# Autodesk Inventor assembly: 1071_assembly
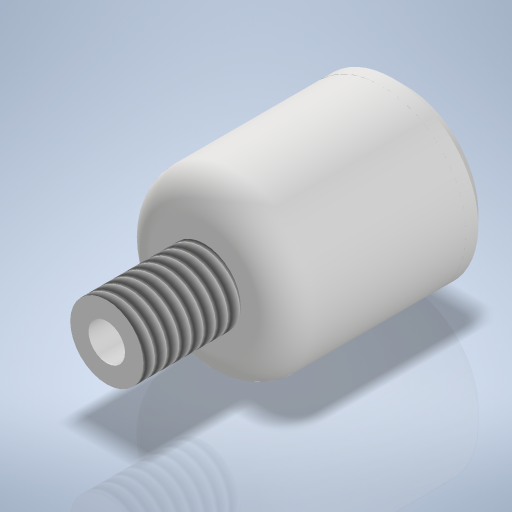
[picture p0: Inventor's stored thumbnail of the model, 512x512]
Saved by Autodesk Inventor 2024 (Build 280153000, 153)
## iProperties
Created: 2024-06-07
Part Number: 1071_assembly
Document SubType Name: Assembly
Designer: ffogue
Author: ffogue
## Documents named in this file (3)
- C:\Users\ffogue\OneDrive - MuM - OM\Dokumente\Inventor\Paddle\1071_assembly.iam
- C:\Users\ffogue\OneDrive - MuM - OM\Dokumente\Inventor\Paddle\1071.ipt
- C:\Users\ffogue\OneDrive - MuM - OM\Dokumente\Inventor\Paddle\1072.ipt
## Components (2 placed, 2 different names)
1. 1071:1 — Einfügen:1
2. 1072:1 — Einfügen:1
## Relationships (1: Insert 1)
- Einfügen:1 [Insert] (-4 mm): 1071:1 ↔ 1072:1
